(part 1 of 2)
# Autodesk Inventor assembly: Motedius_QR-500
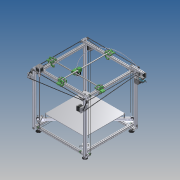
[picture p0: Inventor's stored thumbnail of the model, 180x180]
Saved by Autodesk Inventor 2015 SP1 (Build 190203100, 203)
## iProperties
Created: 2015-01-08
Part Number: Motedius_QR-500
Document SubType Name: Assembly
Designer: Marc
Author: Marc
## Documents named in this file (64)
- E:\Modellflieger\3D Drucker\MotediusQR 500mm\Motedius_QR-500.iam
- E:\Modellflieger\3D Drucker\MotediusQR 500mm\Motedius_20x20_B-Type_Slot-6_500.ipt
- E:\Modellflieger\3D Drucker\MotediusQR 500mm\Motedius_20x20_B-Type_Slot-6_500_MIR.ipt
- E:\Modellflieger\3D Drucker\Eigene Teile\Nema17 Schrittmotor\Nema17_Schrittmotor.iam
- E:\Modellflieger\3D Drucker\Eigene Teile\Nema17 Schrittmotor\Nema17_Montageplatte.ipt
- C:\Users\Marc\Documents\Inventor\Content Center Files\R2015\de-DE\DIN 84\DIN 84 - M3 x 6.ipt
- C:\Users\Marc\Documents\Inventor\Content Center Files\R2015\de-DE\DIN 934\DIN 934 - M6 x 1.ipt
- C:\Users\Marc\Documents\Inventor\Content Center Files\R2015\de-DE\DIN 125-1  A\DIN 125 - A 6,4.ipt
- C:\Users\Marc\Documents\Inventor\Content Center Files\R2015\de-DE\DIN 84\DIN 84 - M6 x 50.ipt
- E:\Modellflieger\3D Drucker\Eigene Teile\Motedis 20 B-Typ Nut 6 Parts\Motedius Gelenkfuß 10 PA\Motedius_Gelenkfuß_10_PA_M6x60.iam
- E:\Modellflieger\3D Drucker\MotediusQR 500mm\Motedius_20x20_B-Type_Slot-6_600.ipt
- E:\Modellflieger\3D Drucker\MotediusQR 500mm\Motedius_20x20_B-Type_Slot-6_290.ipt
- E:\Modellflieger\3D Drucker\MotediusQR 500mm\10mm_Alu_Linearwelle_500mm.ipt
- E:\Modellflieger\3D Drucker\MotediusQR 500mm\X_Y_mit_LM10UU\Lagerblock_Lm10UU.ipt
- E:\Modellflieger\3D Drucker\Eigene Teile\LinearWagen_Mauro_Wheels\Mauro_Wagen_QR_version.iam
- E:\Modellflieger\3D Drucker\Eigene Teile\Linearlager_LM10UU.ipt
- E:\Modellflieger\3D Drucker\Eigene Teile\Openbuilds_Dual_V-Wheel\Openbuilds_Dual_V-Wheel.iam
- E:\Modellflieger\3D Drucker\Eigene Teile\Motedis 20 B-Typ Nut 6 Parts\Motedis_Winkel.ipt
- C:\Users\Marc\Documents\Inventor\Content Center Files\R2015\de-DE\DIN 934\DIN 934 - M5 x 0,8.ipt
- E:\Modellflieger\3D Drucker\Eigene Teile\GT2_20tooth_Pulley\GT2_20tooth.ipt
- E:\Modellflieger\3D Drucker\Eigene Teile\Eigene Schrauben\QR_Ramenschraube_unten_M6x60.iam
- E:\Modellflieger\3D Drucker\Eigene Teile\Eigene Schrauben\QR_Rahmenschraube_oben_M6x80.iam
- E:\Modellflieger\3D Drucker\Eigene Teile\Seilrolle druckbar\Seilrolle.iam
- C:\Users\Marc\Documents\Inventor\Content Center Files\R2015\de-DE\DIN 9021\DIN 9021 - 6,4.ipt
- E:\Modellflieger\3D Drucker\Eigene Teile\Seilrolle druckbar\Distanzscheibe_6x10x0,5mm.ipt
- E:\Modellflieger\3D Drucker\MotediusQR 500mm\Motedius_QR-500\Konstruktions-Assistent\Übertragung des Zahnriemens1.iam
- E:\Modellflieger\3D Drucker\MotediusQR 500mm\Motedius_QR-500\Konstruktions-Assistent\Übertragung des Zahnriemens2.iam
- E:\Modellflieger\3D Drucker\MotediusQR 500mm\Motedius_QR-500\Konstruktions-Assistent\Übertragung des Zahnriemens3.iam
- E:\Modellflieger\3D Drucker\MotediusQR 500mm\Motedius_QR-500\Konstruktions-Assistent\Übertragung des Zahnriemens4.iam
- E:\Modellflieger\3D Drucker\Eigene Teile\Nema17 Schrittmotor\Nema17_Montageplatte_Z-Achse.ipt
- C:\Users\Marc\Documents\Inventor\Content Center Files\R2015\de-DE\DIN 9021\DIN 9021 - 5,3.ipt
- E:\Modellflieger\3D Drucker\MotediusQR 500mm\Importierte Komponenten\Wellenkupplung5-8mm\Wellenkupplung5-8mm.iam
- E:\Modellflieger\3D Drucker\Eigene Teile\Gewindestange_M8x420mm.ipt
- E:\Modellflieger\3D Drucker\MotediusQR 500mm\Gewindestück_M5_Z-Achse.ipt
- E:\Modellflieger\3D Drucker\MotediusQR 500mm\Z-Stage_Wheel_plate.ipt
- E:\Modellflieger\3D Drucker\MotediusQR 500mm\Z-Stage_Wheel_plate_20x20.ipt
- C:\Users\Marc\Documents\Inventor\Content Center Files\R2015\de-DE\DIN 84\DIN 84 - M5 x 30.ipt
- E:\Modellflieger\3D Drucker\Eigene Teile\Eigene Schrauben\Ösenschraube_M3x15.ipt
- C:\Users\Marc\Documents\Inventor\Content Center Files\R2015\de-DE\DIN 934\DIN 934 - M3 x 0,5.ipt
- C:\Users\Marc\Documents\Inventor\Content Center Files\R2015\de-DE\DIN 84\DIN 84 - M5 x 6.ipt
- C:\Users\Marc\Documents\Inventor\Content Center Files\R2015\de-DE\DIN 84\DIN 84 - M5 x 8.ipt
- C:\Users\Marc\Documents\Inventor\Content Center Files\R2015\de-DE\DIN 934\DIN 934 - M8 x 1,25.ipt
- E:\Modellflieger\3D Drucker\MotediusQR 500mm\Z_Stage_Nut_holder_15x15alu.ipt
- C:\Users\Marc\Documents\Inventor\Content Center Files\R2015\de-DE\DIN 84\DIN 84 - M5 x 20.ipt
- E:\Modellflieger\3D Drucker\MotediusQR 500mm\Aluplatte_5mm.ipt
- C:\Users\Marc\Documents\Inventor\Content Center Files\R2015\de-DE\DIN 84\DIN 84 - M5 x 40.ipt
- E:\Modellflieger\3D Drucker\MotediusQR 500mm\Seil1.ipt
- E:\Modellflieger\3D Drucker\MotediusQR 500mm\Seil2.ipt
- E:\Modellflieger\3D Drucker\MotediusQR 500mm\Seil-3.ipt
- E:\Modellflieger\3D Drucker\MotediusQR 500mm\Gewindestück_M5_Z-Achse_55mm.ipt
- E:\Modellflieger\3D Drucker\Eigene Teile\Motedis 20 B-Typ Nut 6 Parts\Motedius_20x20_B-Type_Slot-6_120.ipt
- Motedius_20x20_B-Type_Slot-6_120.ipt
- E:\Modellflieger\3D Drucker\Eigene Teile\POM Extruder\extruder_180Grad.iam
- E:\Modellflieger\3D Drucker\Eigene Teile\Eigene Schrauben\DIN 84 - M6 x 70.ipt
- C:\Users\Marc\Documents\Inventor\Content Center Files\R2015\de-DE\DIN 84\DIN 84 - M5 x 10.ipt
- E:\Modellflieger\3D Drucker\MotediusQR 500mm\Importierte Komponenten\E3D_V6_1.75mm_Universal_HotEnd_Mockup\E3D_V6_1.75mm_Universal_HotEnd_Mockup.ipt
- E:\Modellflieger\3D Drucker\MotediusQR 500mm\Importierte Komponenten\E3D_V6_Fan_Duct\E3D_V6_Fan_Duct.ipt
- E:\Modellflieger\3D Drucker\MotediusQR 500mm\PTFE_Tube_4x2.ipt
- E:\Modellflieger\3D Drucker\MotediusQR 500mm\Importierte Komponenten\12VDC-1.1875-X-0.375-DELTA-BOX-FAN\12VDC-1.1875-X-0.375-DELTA-BOX-FAN.ipt
- C:\Users\Marc\Documents\Inventor\Content Center Files\R2015\de-DE\DIN 84\DIN 84 - M3 x 10.ipt
- C:\Users\Marc\Documents\Inventor\Content Center Files\R2015\de-DE\DIN 84\DIN 84 - M3 x 22.ipt
- C:\Users\Marc\Documents\Inventor\Content Center Files\R2015\de-DE\DIN 84\DIN 84 - M3 x 18.ipt
- E:\Modellflieger\3D Drucker\Eigene Teile\gt2-belt-clamps\gt2_clip_v2.ipt
- C:\Users\Marc\Documents\Inventor\Content Center Files\R2015\de-DE\DIN 84\DIN 84 - M3 x 14.ipt
## Components (294 placed, 59 different names)
1. Motedius_20x20_B-Type_Slot-6_500:1 — Tangential:1, Fluchtend:1, Passend:1, Tangential:3, Fluchtend:3, Passend:3, Passend:5, Passend:7, Passend:9, Passend:79, Passend:89, Fluchtend:55
2. Motedius_20x20_B-Type_Slot-6_500:2 — Tangential:1, Fluchtend:1, Passend:1, Tangential:2, Passend:2, Fluchtend:2, Fluchtend:5, Passend:10, Passend:13, Fluchtend:7, Einfügen:30, Einfügen:32, Fluchtend:44
3. Motedius_20x20_B-Type_Slot-6_500:3 — Tangential:2, Passend:2, Fluchtend:2, Passend:11, Passend:14, Passend:91, Passend:93, Passend:137, Fluchtend:45
4. Motedius_20x20_B-Type_Slot-6_500:4 — Tangential:3, Fluchtend:3, Passend:3, Passend:4, Passend:6, Fluchtend:4, Passend:8, Passend:12, Fluchtend:6, Einfügen:29, Einfügen:31, Fluchtend:31, Fluchtend:54
5. Motedius_20x20_B-Type_Slot-6_500:5 — Passend:7, Fluchtend:4, Passend:8, Passend:20, Fluchtend:12, Einfügen:71, Einfügen:72, Einfügen:86, Einfügen:87
6. Motedius_20x20_B-Type_Slot-6_500:6 — Passend:9, Fluchtend:5, Passend:10, Passend:23, Fluchtend:13, Einfügen:76, Einfügen:77, Einfügen:79, Einfügen:80
7. Motedius_20x20_B-Type_Slot-6_500:7 — Passend:13, Passend:14, Fluchtend:7, Passend:25, Fluchtend:14, Einfügen:75, Einfügen:78
8. Motedius_20x20_B-Type_Slot-6_500:8 — Passend:11, Passend:12, Fluchtend:6, Passend:27, Fluchtend:15, Einfügen:73, Einfügen:74, Einfügen:88, Einfügen:89
9. Motedius_20x20_B-Type_Slot-6_500_MIR:1 — Passend:15, Passend:16, Fluchtend:8, Tangential:4, Passend:19, Fluchtend:11, Tangential:6, Passend:21, Passend:22, Einfügen:26, Einfügen:27, Passend:163, Passend:164
10. Motedius_20x20_B-Type_Slot-6_500_MIR:2 — Passend:16, Fluchtend:8, Tangential:4, Fluchtend:9, Passend:17, Tangential:5, Passend:67, Passend:165, Passend:166, Passend:262, Fluchtend:62, Passend:263
11. Motedius_20x20_B-Type_Slot-6_500_MIR:3 — Fluchtend:9, Passend:17, Tangential:5, Passend:24, Passend:26, Einfügen:25, Einfügen:28, Passend:159, Passend:160
12. Motedius_20x20_B-Type_Slot-6_500_MIR:4 — Passend:18, Fluchtend:10, Passend:19, Fluchtend:11, Tangential:6, Passend:63, Passend:65, Passend:161, Passend:162, Passend:175, Fluchtend:34, Fluchtend:35
13. Nema17_Schrittmotor:1 [sub-assembly] — Einfügen:1, Tangential:7, Einfügen:2, Einfügen:3, Einfügen:4, Einfügen:5, Einfügen:66
14. Nema17_Montageplatte:1 — Einfügen:1, Tangential:7, Passend:20, Fluchtend:12, Passend:21
15. DIN 84 - ersetzt durch DIN EN ISO 1207 M3 x 6:1 — Einfügen:2
16. DIN 84 - ersetzt durch DIN EN ISO 1207 M3 x 6:2 — Einfügen:5
17. DIN 84 - ersetzt durch DIN EN ISO 1207 M3 x 6:3 — Einfügen:3
18. DIN 84 - ersetzt durch DIN EN ISO 1207 M3 x 6:4 — Einfügen:4
19. Nema17_Schrittmotor:2 [sub-assembly] — Einfügen:67
20. Nema17_Montageplatte:2 — Passend:22, Passend:23, Fluchtend:13
21. DIN 84 - ersetzt durch DIN EN ISO 1207 M3 x 6:5
22. DIN 84 - ersetzt durch DIN EN ISO 1207 M3 x 6:6
23. DIN 84 - ersetzt durch DIN EN ISO 1207 M3 x 6:7
24. DIN 84 - ersetzt durch DIN EN ISO 1207 M3 x 6:8
25. Nema17_Schrittmotor:3 [sub-assembly] — Einfügen:68
26. Nema17_Montageplatte:3 — Passend:24, Passend:25, Fluchtend:14
27. DIN 84 - ersetzt durch DIN EN ISO 1207 M3 x 6:9
28. DIN 84 - ersetzt durch DIN EN ISO 1207 M3 x 6:10
29. DIN 84 - ersetzt durch DIN EN ISO 1207 M3 x 6:11
30. DIN 84 - ersetzt durch DIN EN ISO 1207 M3 x 6:12
31. Nema17_Schrittmotor:4 [sub-assembly] — Einfügen:65
32. Nema17_Montageplatte:4 — Passend:26, Passend:27, Fluchtend:15
33. DIN 84 - ersetzt durch DIN EN ISO 1207 M3 x 6:13
34. DIN 84 - ersetzt durch DIN EN ISO 1207 M3 x 6:14
35. DIN 84 - ersetzt durch DIN EN ISO 1207 M3 x 6:15
36. DIN 84 - ersetzt durch DIN EN ISO 1207 M3 x 6:16
37. DIN 84 - ersetzt durch DIN EN ISO 1207 M6 x 50:1 — Passend:52, Passend:53, Passend:62, Passend:70
38. DIN 125-1 A A 6,4:9 — Passend:52, Passend:53, Einfügen:25
39. DIN 84 - M6 x 70:1 — Passend:265, Passend:267
40. DIN 125-1 A A 6,4:10 — Einfügen:28
41. DIN 84 - ersetzt durch DIN EN ISO 1207 M6 x 50:3 — Passend:64, Passend:72
42. DIN 125-1 A A 6,4:11 — Einfügen:26
43. DIN 84 - ersetzt durch DIN EN ISO 1207 M6 x 50:4 — Passend:66, Passend:74
44. DIN 125-1 A A 6,4:12 — Einfügen:27
45. DIN 125-1 A A 6,4:14 — Passend:62, Passend:63, Passend:71
46. DIN 125-1 A A 6,4:15 — Passend:64, Passend:65, Passend:73
47. DIN 125-1 A A 6,4:16 — Passend:66, Passend:67, Passend:75
48. DIN 934 - ersetzt durch DIN EN 24032/28673/28674 M6:6 — Passend:70, Passend:71
49. DIN 934 - ersetzt durch DIN EN 24032/28673/28674 M6:7 — Passend:72, Passend:73
50. DIN 934 - ersetzt durch DIN EN 24032/28673/28674 M6:8 — Passend:74, Passend:75
51. Motedius_Gelenkfuß_10_PA_M6x60:1 [sub-assembly] — Passend:76, Passend:77, Passend:78, Passend:80
52. DIN 125-1 A A 6,4:17 — Passend:76, Passend:77, Einfügen:29
53. DIN 125-1 A A 6,4:18 — Passend:78, Passend:79, Passend:81
54. DIN 934 - ersetzt durch DIN EN 24032/28673/28674 M6:9 — Passend:80, Passend:81
55. Motedius_Gelenkfuß_10_PA_M6x60:2 [sub-assembly] — Passend:88, Passend:94
56. DIN 125-1 A A 6,4:19 — Einfügen:30
57. Motedius_Gelenkfuß_10_PA_M6x60:3 [sub-assembly] — Passend:92, Passend:98
58. DIN 125-1 A A 6,4:20 — Einfügen:31
59. Motedius_Gelenkfuß_10_PA_M6x60:4 [sub-assembly] — Passend:90, Passend:96
60. DIN 125-1 A A 6,4:21 — Einfügen:32
61. DIN 125-1 A A 6,4:22 — Passend:88, Passend:89, Passend:95
62. DIN 125-1 A A 6,4:23 — Passend:90, Passend:91, Passend:97
63. DIN 125-1 A A 6,4:24 — Passend:92, Passend:93, Passend:99
64. DIN 934 - ersetzt durch DIN EN 24032/28673/28674 M6:10 — Passend:94, Passend:95
65. DIN 934 - ersetzt durch DIN EN 24032/28673/28674 M6:11 — Passend:96, Passend:97
66. DIN 934 - ersetzt durch DIN EN 24032/28673/28674 M6:12 — Passend:98, Passend:99
67. Motedius_20x20_B-Type_Slot-6_600:1 — Passend:135, Fluchtend:23, Fluchtend:24, Fluchtend:25, Passend:136, Fluchtend:26, Passend:137, Fluchtend:27, Passend:138, Passend:141, Passend:142, Passend:144, Fluchtend:29, Passend:196, Fluchtend:40, Fluchtend:41, Fluchtend:42, Passend:197, Passend:202, Fluchtend:46, Fluchtend:47, Passend:203, Fluchtend:48, Passend:235, Passend:237, Passend:243
68. Motedius_20x20_B-Type_Slot-6_290:1 — Passend:135, Fluchtend:23, Fluchtend:24, Passend:140, Passend:145, Passend:186, Fluchtend:36, Fluchtend:37, Passend:187, Fluchtend:38, Fluchtend:39, Passend:232, Passend:241
69. Motedius_20x20_B-Type_Slot-6_290:2 — Fluchtend:25, Passend:136, Fluchtend:26, Passend:139, Passend:143, Fluchtend:28, Fluchtend:50, Passend:210, Fluchtend:51, Passend:211, Fluchtend:52, Passend:239
70. Openbuilds_Dual_V-Wheel:5 [sub-assembly] — Einfügen:155
71. Openbuilds_Dual_V-Wheel:6 [sub-assembly] — Einfügen:153
72. Openbuilds_Dual_V-Wheel:7 [sub-assembly] — Einfügen:157
73. Openbuilds_Dual_V-Wheel:8 [sub-assembly] — Einfügen:150
74. Motedis_Winkel:9 — Fluchtend:27, Passend:138, Passend:139, Fluchtend:45, Einfügen:179, Einfügen:180
75. Motedis_Winkel:10 — Passend:140, Passend:141, Fluchtend:31, Einfügen:177, Einfügen:178
76. Motedis_Winkel:11 — Passend:142, Passend:143, Fluchtend:28, Fluchtend:44, Einfügen:181, Einfügen:182
77. Motedis_Winkel:12 — Passend:144, Passend:145, Fluchtend:29, Einfügen:183, Einfügen:184
78. Mauro_Wagen_QR_version:5 [sub-assembly] — Passend:159, Passend:160, Fluchtend:33, Passend:289, Fluchtend:73, Fluchtend:74, Einfügen:203
79. Mauro_Wagen_QR_version:6 [sub-assembly] — Passend:161, Passend:162, Fluchtend:32, Passend:287, Fluchtend:69, Fluchtend:70, Einfügen:204
80. Mauro_Wagen_QR_version:7 [sub-assembly] — Passend:165, Passend:166, Fluchtend:32, Einfügen:48, Passend:288, Fluchtend:71, Fluchtend:72, Einfügen:206
81. Mauro_Wagen_QR_version:8 [sub-assembly] — Passend:163, Passend:164, Fluchtend:33, Einfügen:47, Passend:285, Fluchtend:67, Fluchtend:68, Passend:286, Einfügen:205
82. 10mm_Alu_Linearwelle_500mm:1 — Einfügen:47, Einfügen:52
83. 10mm_Alu_Linearwelle_500mm:2 — Einfügen:48, Einfügen:51
84. Lagerblock_Lm10UU:1 — Einfügen:49, Einfügen:50, Einfügen:51, Einfügen:52, Einfügen:195, Einfügen:197, Einfügen:198, Passend:274, Passend:276, Einfügen:199, Einfügen:200, Passend:278, Passend:280, Einfügen:201, Einfügen:202, Passend:282, Passend:284
85. Linearlager_LM10UU:1 — Einfügen:50
86. Linearlager_LM10UU:2 — Einfügen:49
87. QR_Rahmenschraube_oben_M6x80:2 [sub-assembly] — Einfügen:75
88. QR_Rahmenschraube_oben_M6x80:3 [sub-assembly] — Einfügen:72
89. QR_Rahmenschraube_oben_M6x80:4 [sub-assembly] — Einfügen:73
90. QR_Rahmenschraube_oben_M6x80:5 [sub-assembly] — Einfügen:77, Einfügen:111
91. QR_Rahmenschraube_oben_M6x80:6 [sub-assembly] — Einfügen:74, Einfügen:135
92. QR_Rahmenschraube_oben_M6x80:7 [sub-assembly] — Einfügen:76
93. QR_Rahmenschraube_oben_M6x80:8 [sub-assembly] — Einfügen:71
94. DIN 84 - ersetzt durch DIN EN ISO 1207 M5 x 30:2 — Einfügen:156, Passend:212, Passend:214, Passend:216
95. DIN 84 - ersetzt durch DIN EN ISO 1207 M5 x 30:1 — Passend:169, Einfügen:151, Passend:198, Passend:200
96. DIN 934 - ersetzt durch DIN EN 24032/28673/28674 M5:2 — Passend:169, Einfügen:152
97. GT2_20tooth:1 — Einfügen:65
98. GT2_20tooth:2 — Einfügen:66
99. GT2_20tooth:3 — Einfügen:67
100. GT2_20tooth:4 — Einfügen:68
101. QR_Ramenschraube_unten_M6x60:1 [sub-assembly] — Einfügen:147
102. QR_Rahmenschraube_oben_M6x80:1 [sub-assembly] — Einfügen:148
103. QR_Ramenschraube_unten_M6x60:2 [sub-assembly] — Einfügen:78
104. QR_Ramenschraube_unten_M6x60:3 [sub-assembly] — Einfügen:80
105. QR_Ramenschraube_unten_M6x60:4 [sub-assembly] — Einfügen:79, Einfügen:81, Passend:176
106. Seilrolle:1 [sub-assembly] — Einfügen:83, Einfügen:84
107. DIN 9021 6,4:1 — Einfügen:81, Einfügen:82
108. DIN 9021 6,4:2 — Einfügen:85, Passend:177
109. Distanzscheibe_6x10x0,5mm:1 — Einfügen:82, Einfügen:83
110. Distanzscheibe_6x10x0,5mm:2 — Einfügen:84, Einfügen:85
111. QR_Ramenschraube_unten_M6x60:5 [sub-assembly] — Einfügen:87, Einfügen:123
112. QR_Ramenschraube_unten_M6x60:6 [sub-assembly] — Einfügen:86, Einfügen:117
113. QR_Ramenschraube_unten_M6x60:7 [sub-assembly] — Einfügen:89, Einfügen:129
114. QR_Ramenschraube_unten_M6x60:8 [sub-assembly] — Einfügen:88, Einfügen:141
115. Übertragung des Zahnriemens:1 [sub-assembly]
116. Übertragung des Zahnriemens:2 [sub-assembly]
117. Übertragung des Zahnriemens:3 [sub-assembly]
118. Übertragung des Zahnriemens:4 [sub-assembly]
119. Nema17_Schrittmotor:5 [sub-assembly] — Einfügen:99
120. Nema17_Montageplatte_Z-Achse:1 — Passend:175, Fluchtend:34, Fluchtend:35, Einfügen:95, Einfügen:97, Einfügen:193, Einfügen:194
121. DIN 84 - ersetzt durch DIN EN ISO 1207 M3 x 6:17
122. DIN 84 - ersetzt durch DIN EN ISO 1207 M3 x 6:18
123. DIN 84 - ersetzt durch DIN EN ISO 1207 M3 x 6:19
124. DIN 84 - ersetzt durch DIN EN ISO 1207 M3 x 6:20
125. DIN 9021 5,3:1 — Einfügen:95, Einfügen:96
126. DIN 9021 5,3:2 — Einfügen:96
127. DIN 9021 5,3:3 — Einfügen:98
128. DIN 9021 5,3:4 — Einfügen:97, Einfügen:98
129. Wellenkupplung5-8mm:1 [sub-assembly] — Einfügen:99, Einfügen:100
130. Gewindestange_M8x420mm:1 — Einfügen:100, Tangential:12
131. DIN 934 - ersetzt durch DIN EN 24032/28673/28674 M6:13 — Passend:176, Passend:177
132. Seilrolle:2 [sub-assembly]
133. DIN 9021 6,4:3 — Einfügen:111
134. DIN 9021 6,4:4 — Einfügen:105
135. Distanzscheibe_6x10x0,5mm:3
136. Distanzscheibe_6x10x0,5mm:4
137. DIN 934 - ersetzt durch DIN EN 24032/28673/28674 M6:14 — Einfügen:105
138. Seilrolle:3 [sub-assembly]
139. DIN 9021 6,4:5 — Einfügen:117
140. DIN 9021 6,4:6
141. Distanzscheibe_6x10x0,5mm:5
142. Distanzscheibe_6x10x0,5mm:6
143. DIN 934 - ersetzt durch DIN EN 24032/28673/28674 M6:15
144. Seilrolle:4 [sub-assembly] — Fluchtend:56
145. DIN 9021 6,4:7 — Einfügen:123
146. DIN 9021 6,4:8
147. Distanzscheibe_6x10x0,5mm:7
148. Distanzscheibe_6x10x0,5mm:8
149. DIN 934 - ersetzt durch DIN EN 24032/28673/28674 M6:16
150. Seilrolle:5 [sub-assembly]
151. DIN 9021 6,4:9 — Einfügen:129
152. DIN 9021 6,4:10
153. Distanzscheibe_6x10x0,5mm:9
154. Distanzscheibe_6x10x0,5mm:10
155. DIN 934 - ersetzt durch DIN EN 24032/28673/28674 M6:17
156. Seilrolle:6 [sub-assembly]
157. DIN 9021 6,4:11 — Einfügen:135
158. DIN 9021 6,4:12
159. Distanzscheibe_6x10x0,5mm:11
160. Distanzscheibe_6x10x0,5mm:12
161. DIN 934 - ersetzt durch DIN EN 24032/28673/28674 M6:18
162. Seilrolle:7 [sub-assembly] — Fluchtend:59
163. DIN 9021 6,4:13 — Einfügen:141
164. DIN 9021 6,4:14
165. Distanzscheibe_6x10x0,5mm:13
166. Distanzscheibe_6x10x0,5mm:14
167. DIN 934 - ersetzt durch DIN EN 24032/28673/28674 M6:19
168. Seilrolle:8 [sub-assembly]
169. DIN 9021 6,4:15 — Einfügen:147
170. DIN 9021 6,4:16
171. Distanzscheibe_6x10x0,5mm:15
172. Distanzscheibe_6x10x0,5mm:16
173. DIN 934 - ersetzt durch DIN EN 24032/28673/28674 M6:20
174. Seilrolle:9 [sub-assembly]
175. DIN 9021 6,4:17 — Einfügen:148
176. DIN 9021 6,4:18
177. Distanzscheibe_6x10x0,5mm:17
178. Distanzscheibe_6x10x0,5mm:18
179. DIN 934 - ersetzt durch DIN EN 24032/28673/28674 M6:21
180. Gewindestück_M5_Z-Achse:1 — Einfügen:149, Passend:188, Passend:190, Passend:192, Passend:194
181. Z-Stage_Wheel_plate:1 — Passend:186, Fluchtend:36, Fluchtend:37, Einfügen:149, Einfügen:150, Passend:189, Passend:193, Einfügen:173, Einfügen:174
182. Z-Stage_Wheel_plate:2 — Passend:187, Fluchtend:38, Fluchtend:39, Passend:191, Passend:195, Einfügen:171, Einfügen:172
183. DIN 934 - ersetzt durch DIN EN 24032/28673/28674 M5:5 — Passend:188, Passend:189
184. DIN 934 - ersetzt durch DIN EN 24032/28673/28674 M5:6 — Passend:190, Passend:191
185. DIN 934 - ersetzt durch DIN EN 24032/28673/28674 M5:7 — Passend:192, Passend:193
186. DIN 934 - ersetzt durch DIN EN 24032/28673/28674 M5:8 — Passend:194, Passend:195
187. Z-Stage_Wheel_plate_20x20:1 — Fluchtend:42, Passend:197, Fluchtend:43, Einfügen:152, Passend:201, Einfügen:169, Einfügen:170
188. Z-Stage_Wheel_plate_20x20:2 — Passend:196, Fluchtend:40, Fluchtend:41, Fluchtend:43, Einfügen:151, Einfügen:153, Passend:199, Einfügen:158, Passend:219, Passend:221, Einfügen:167, Einfügen:168
189. DIN 934 - ersetzt durch DIN EN 24032/28673/28674 M5:9 — Passend:198, Passend:199
190. DIN 934 - ersetzt durch DIN EN 24032/28673/28674 M5:10 — Passend:200, Passend:201
191. Z-Stage_Wheel_plate_20x20:3 — Passend:202, Fluchtend:46, Fluchtend:47, Fluchtend:49, Passend:205, Einfügen:159, Passend:227, Passend:229, Einfügen:161, Einfügen:162, Einfügen:192, Passend:261
192. Z-Stage_Wheel_plate:3 — Passend:203, Fluchtend:48, Fluchtend:49, Einfügen:155, Passend:207, Passend:209, Einfügen:175, Einfügen:176
193. Gewindestück_M5_Z-Achse_55mm:1 — Einfügen:192, Passend:260
194. DIN 934 - ersetzt durch DIN EN 24032/28673/28674 M5:11 — Passend:205
195. DIN 934 - ersetzt durch DIN EN 24032/28673/28674 M5:12 — Passend:207
196. DIN 934 - ersetzt durch DIN EN 24032/28673/28674 M5:13 — Passend:209
197. Z-Stage_Wheel_plate_20x20:4 — Fluchtend:50, Passend:210, Fluchtend:51, Fluchtend:53, Einfügen:156, Einfügen:157, Passend:215, Einfügen:160, Passend:223, Passend:225, Einfügen:165, Einfügen:166
198. Z-Stage_Wheel_plate_20x20:5 — Passend:211, Fluchtend:52, Fluchtend:53, Passend:213, Passend:217, Einfügen:163, Einfügen:164
199. DIN 934 - ersetzt durch DIN EN 24032/28673/28674 M5:14 — Passend:212, Passend:213
200. DIN 934 - ersetzt durch DIN EN 24032/28673/28674 M5:15 — Passend:214, Passend:215
201. DIN 934 - ersetzt durch DIN EN 24032/28673/28674 M5:16 — Passend:216, Passend:217
202. Ösenschraube_M3x15:1 — Einfügen:158, Passend:218, Passend:220
203. DIN 934 - ersetzt durch DIN EN 24032/28673/28674 M3:1 — Passend:218, Passend:219
204. DIN 934 - ersetzt durch DIN EN 24032/28673/28674 M3:2 — Passend:220, Passend:221
205. Ösenschraube_M3x15:2 — Einfügen:159, Passend:226, Passend:228
206. Ösenschraube_M3x15:3 — Einfügen:160, Passend:222, Passend:224
207. DIN 934 - ersetzt durch DIN EN 24032/28673/28674 M3:3 — Passend:222, Passend:223
208. DIN 934 - ersetzt durch DIN EN 24032/28673/28674 M3:4 — Passend:224, Passend:225
209. DIN 934 - ersetzt durch DIN EN 24032/28673/28674 M3:5 — Passend:226, Passend:227
210. DIN 934 - ersetzt durch DIN EN 24032/28673/28674 M3:6 — Passend:228, Passend:229
211. DIN 84 - ersetzt durch DIN EN ISO 1207 M5 x 6:1 — Einfügen:161
212. DIN 84 - ersetzt durch DIN EN ISO 1207 M5 x 6:2 — Einfügen:162
213. DIN 84 - ersetzt durch DIN EN ISO 1207 M5 x 6:3 — Einfügen:164
214. DIN 84 - ersetzt durch DIN EN ISO 1207 M5 x 6:4 — Einfügen:163
215. DIN 84 - ersetzt durch DIN EN ISO 1207 M5 x 6:5 — Einfügen:165
216. DIN 84 - ersetzt durch DIN EN ISO 1207 M5 x 6:6 — Einfügen:166
217. DIN 84 - ersetzt durch DIN EN ISO 1207 M5 x 6:7 — Einfügen:167
218. DIN 84 - ersetzt durch DIN EN ISO 1207 M5 x 6:8 — Einfügen:168
219. DIN 84 - ersetzt durch DIN EN ISO 1207 M5 x 6:9 — Einfügen:169
220. DIN 84 - ersetzt durch DIN EN ISO 1207 M5 x 6:10 — Einfügen:170
221. DIN 84 - ersetzt durch DIN EN ISO 1207 M5 x 6:11 — Einfügen:171
222. DIN 84 - ersetzt durch DIN EN ISO 1207 M5 x 6:12 — Einfügen:172
223. DIN 84 - ersetzt durch DIN EN ISO 1207 M5 x 6:13 — Einfügen:173
224. DIN 84 - ersetzt durch DIN EN ISO 1207 M5 x 6:14 — Einfügen:174
225. DIN 84 - ersetzt durch DIN EN ISO 1207 M5 x 6:15 — Einfügen:175
226. DIN 84 - ersetzt durch DIN EN ISO 1207 M5 x 6:16 — Einfügen:176
227. DIN 84 - ersetzt durch DIN EN ISO 1207 M5 x 8:1 — Einfügen:178
228. DIN 84 - ersetzt durch DIN EN ISO 1207 M5 x 8:2 — Einfügen:177
229. DIN 84 - ersetzt durch DIN EN ISO 1207 M5 x 8:3 — Einfügen:179
230. DIN 84 - ersetzt durch DIN EN ISO 1207 M5 x 8:4 — Einfügen:180
231. DIN 84 - ersetzt durch DIN EN ISO 1207 M5 x 8:5 — Einfügen:181
232. DIN 84 - ersetzt durch DIN EN ISO 1207 M5 x 8:6 — Einfügen:182
233. DIN 84 - ersetzt durch DIN EN ISO 1207 M5 x 8:7 — Einfügen:183
234. DIN 84 - ersetzt durch DIN EN ISO 1207 M5 x 8:8 — Einfügen:184
235. DIN 934 - ersetzt durch DIN EN 24032/28673/28674 M8:1 — Einfügen:185, Passend:230, Tangential:12
236. Z_Stage_Nut_holder_15x15alu:1 — Einfügen:185, Passend:230, Einfügen:186, Passend:231, Passend:232, Einfügen:187
237. DIN 934 - ersetzt durch DIN EN 24032/28673/28674 M8:2 — Einfügen:186, Passend:231
238. DIN 84 - ersetzt durch DIN EN ISO 1207 M5 x 20:1 — Passend:233, Passend:234
239. DIN 9021 5,3:5 — Passend:233, Passend:234, Einfügen:187
240. Aluplatte_5mm:1 — Einfügen:188, Einfügen:189, Einfügen:190, Einfügen:191, Fluchtend:54, Fluchtend:55, Passend:253, Passend:255, Passend:257, Passend:259
241. DIN 84 - ersetzt durch DIN EN ISO 1207 M5 x 40:2 — Einfügen:189, Passend:238, Passend:250, Passend:256
242. DIN 84 - ersetzt durch DIN EN ISO 1207 M5 x 40:3 — Einfügen:188, Passend:235, Passend:236, Passend:244, Passend:258
243. DIN 84 - ersetzt durch DIN EN ISO 1207 M5 x 40:4 — Einfügen:190, Passend:240, Passend:248, Passend:252
244. DIN 84 - ersetzt durch DIN EN ISO 1207 M5 x 40:5 — Einfügen:191, Passend:242, Passend:246, Passend:254
245. DIN 9021 5,3:6 — Passend:236, Passend:237, Passend:245
246. DIN 9021 5,3:7 — Passend:238, Passend:239, Passend:251
247. DIN 9021 5,3:8 — Passend:240, Passend:241, Passend:249
248. DIN 9021 5,3:9 — Passend:242, Passend:243, Passend:247
249. DIN 934 - ersetzt durch DIN EN 24032/28673/28674 M5:17 — Passend:244, Passend:245
250. DIN 934 - ersetzt durch DIN EN 24032/28673/28674 M5:18 — Passend:246, Passend:247
251. DIN 934 - ersetzt durch DIN EN 24032/28673/28674 M5:19 — Passend:248, Passend:249
252. DIN 934 - ersetzt durch DIN EN 24032/28673/28674 M5:20 — Passend:250, Passend:251
253. DIN 934 - ersetzt durch DIN EN 24032/28673/28674 M5:21 — Passend:252, Passend:253
254. DIN 934 - ersetzt durch DIN EN 24032/28673/28674 M5:22 — Passend:254, Passend:255
255. DIN 934 - ersetzt durch DIN EN 24032/28673/28674 M5:23 — Passend:256, Passend:257
256. DIN 934 - ersetzt durch DIN EN 24032/28673/28674 M5:24 — Passend:258, Passend:259
257. Seil1:1
258. Seil2:1 — Fluchtend:57, Fluchtend:58
259. Seil-3:1 — Fluchtend:60, Fluchtend:61
260. DIN 934 - ersetzt durch DIN EN 24032/28673/28674 M5:25 — Passend:260, Passend:261
261. Motedius_20x20_B-Type_Slot-6_120:1 — Passend:262, Fluchtend:62, Passend:263, Passend:264, Fluchtend:63, Fluchtend:64, Passend:266
262. extruder_180Grad:1 [sub-assembly] — Passend:264, Fluchtend:63, Fluchtend:64, Passend:270
263. DIN 9021 6,4:19 — Passend:265, Passend:266, Passend:268
264. DIN 934 - ersetzt durch DIN EN 24032/28673/28674 M6:22 — Passend:267, Passend:268
265. DIN 84 - ersetzt durch DIN EN ISO 1207 M5 x 10:1 — Einfügen:193
266. DIN 84 - ersetzt durch DIN EN ISO 1207 M5 x 10:2 — Einfügen:194
267. E3D_V6_1.75mm_Universal_HotEnd_Mockup:1 — Einfügen:195, Tangential:13, Passend:269, Fluchtend:66
268. E3D_V6_Fan_Duct:1 — Tangential:13, Einfügen:196
269. PTFE_Tube_4x2:1 — Fluchtend:65, Fluchtend:66
270. 12VDC-1.1875-X-0.375-DELTA-BOX-FAN:1 — Einfügen:196
271. DIN 84 - ersetzt durch DIN EN ISO 1207 M3 x 10:1 — Einfügen:197, Passend:273
272. DIN 84 - ersetzt durch DIN EN ISO 1207 M3 x 10:2 — Einfügen:198, Passend:275
273. DIN 934 - ersetzt durch DIN EN 24032/28673/28674 M3:7 — Passend:273, Passend:274
274. DIN 934 - ersetzt durch DIN EN 24032/28673/28674 M3:8 — Passend:275, Passend:276
275. DIN 84 - ersetzt durch DIN EN ISO 1207 M3 x 22:1 — Einfügen:200, Passend:277
276. DIN 84 - ersetzt durch DIN EN ISO 1207 M3 x 22:2 — Einfügen:199, Passend:279
277. DIN 934 - ersetzt durch DIN EN 24032/28673/28674 M3:9 — Passend:277, Passend:278
278. DIN 934 - ersetzt durch DIN EN 24032/28673/28674 M3:10 — Passend:279, Passend:280
279. DIN 84 - ersetzt durch DIN EN ISO 1207 M3 x 18:1 — Einfügen:202, Passend:283
280. DIN 84 - ersetzt durch DIN EN ISO 1207 M3 x 18:2 — Einfügen:201, Passend:281
281. DIN 934 - ersetzt durch DIN EN 24032/28673/28674 M3:11 — Passend:281, Passend:282
282. DIN 934 - ersetzt durch DIN EN 24032/28673/28674 M3:12 — Passend:283, Passend:284
283. gt2_clip_v2:1 — Passend:285, Fluchtend:67, Fluchtend:68, Passend:286, Passend:295
284. gt2_clip_v2:2 — Passend:289, Fluchtend:73, Fluchtend:74, Passend:291
285. gt2_clip_v2:3 — Passend:288, Fluchtend:71, Fluchtend:72, Passend:297
286. gt2_clip_v2:4 — Passend:287, Fluchtend:69, Fluchtend:70, Passend:293
287. DIN 84 - ersetzt durch DIN EN ISO 1207 M3 x 14:1 — Einfügen:203, Passend:290
288. DIN 84 - ersetzt durch DIN EN ISO 1207 M3 x 14:2 — Einfügen:204, Passend:292
289. DIN 84 - ersetzt durch DIN EN ISO 1207 M3 x 14:3 — Einfügen:205, Passend:294
290. DIN 84 - ersetzt durch DIN EN ISO 1207 M3 x 14:4 — Einfügen:206, Passend:296
291. DIN 934 - ersetzt durch DIN EN 24032/28673/28674 M3:13 — Passend:290, Passend:291
292. DIN 934 - ersetzt durch DIN EN 24032/28673/28674 M3:14 — Passend:292, Passend:293
293. DIN 934 - ersetzt durch DIN EN 24032/28673/28674 M3:15 — Passend:294, Passend:295
294. DIN 934 - ersetzt durch DIN EN 24032/28673/28674 M3:16 — Passend:296, Passend:297
## Relationships (476: Mate 214, Insert 183, Flush 66, Tangent 13)
- Tangential:1: Motedius_20x20_B-Type_Slot-6_500:1 ↔ Motedius_20x20_B-Type_Slot-6_500:2
- Fluchtend:1 [Flush] (20 mm): Motedius_20x20_B-Type_Slot-6_500:1 ↔ Motedius_20x20_B-Type_Slot-6_500:2
- Passend:1 [Mate]: Motedius_20x20_B-Type_Slot-6_500:1 ↔ Motedius_20x20_B-Type_Slot-6_500:2
- Tangential:2: Motedius_20x20_B-Type_Slot-6_500:2 ↔ Motedius_20x20_B-Type_Slot-6_500:3
- Passend:2 [Mate]: Motedius_20x20_B-Type_Slot-6_500:2 ↔ Motedius_20x20_B-Type_Slot-6_500:3
- Fluchtend:2 [Flush] (-20 mm): Motedius_20x20_B-Type_Slot-6_500:2 ↔ Motedius_20x20_B-Type_Slot-6_500:3
- Tangential:3: Motedius_20x20_B-Type_Slot-6_500:1 ↔ Motedius_20x20_B-Type_Slot-6_500:4
- Fluchtend:3 [Flush] (-20 mm): Motedius_20x20_B-Type_Slot-6_500:1 ↔ Motedius_20x20_B-Type_Slot-6_500:4
- Passend:3 [Mate]: Motedius_20x20_B-Type_Slot-6_500:1 ↔ Motedius_20x20_B-Type_Slot-6_500:4
- Passend:4 [Mate] (-250 mm): Motedius_20x20_B-Type_Slot-6_500:4
- Passend:5 [Mate] (-250 mm): Motedius_20x20_B-Type_Slot-6_500:1
- Passend:6 [Mate] (-250 mm): Motedius_20x20_B-Type_Slot-6_500:4
- Passend:7 [Mate]: Motedius_20x20_B-Type_Slot-6_500:1 ↔ Motedius_20x20_B-Type_Slot-6_500:5
- Fluchtend:4 [Flush]: Motedius_20x20_B-Type_Slot-6_500:4 ↔ Motedius_20x20_B-Type_Slot-6_500:5
- Passend:8 [Mate]: Motedius_20x20_B-Type_Slot-6_500:4 ↔ Motedius_20x20_B-Type_Slot-6_500:5
- Passend:9 [Mate]: Motedius_20x20_B-Type_Slot-6_500:1 ↔ Motedius_20x20_B-Type_Slot-6_500:6
- Fluchtend:5 [Flush]: Motedius_20x20_B-Type_Slot-6_500:2 ↔ Motedius_20x20_B-Type_Slot-6_500:6
- Passend:10 [Mate]: Motedius_20x20_B-Type_Slot-6_500:2 ↔ Motedius_20x20_B-Type_Slot-6_500:6
- Passend:11 [Mate]: Motedius_20x20_B-Type_Slot-6_500:3 ↔ Motedius_20x20_B-Type_Slot-6_500:8
- Passend:12 [Mate]: Motedius_20x20_B-Type_Slot-6_500:4 ↔ Motedius_20x20_B-Type_Slot-6_500:8
- Fluchtend:6 [Flush]: Motedius_20x20_B-Type_Slot-6_500:4 ↔ Motedius_20x20_B-Type_Slot-6_500:8
- Passend:13 [Mate]: Motedius_20x20_B-Type_Slot-6_500:2 ↔ Motedius_20x20_B-Type_Slot-6_500:7
- Passend:14 [Mate]: Motedius_20x20_B-Type_Slot-6_500:3 ↔ Motedius_20x20_B-Type_Slot-6_500:7
- Fluchtend:7 [Flush]: Motedius_20x20_B-Type_Slot-6_500:2 ↔ Motedius_20x20_B-Type_Slot-6_500:7
- Passend:15 [Mate] (-250 mm): Motedius_20x20_B-Type_Slot-6_500_MIR:1
- Passend:16 [Mate]: Motedius_20x20_B-Type_Slot-6_500_MIR:1 ↔ Motedius_20x20_B-Type_Slot-6_500_MIR:2
- Fluchtend:8 [Flush] (20 mm): Motedius_20x20_B-Type_Slot-6_500_MIR:1 ↔ Motedius_20x20_B-Type_Slot-6_500_MIR:2
- Tangential:4: Motedius_20x20_B-Type_Slot-6_500_MIR:1 ↔ Motedius_20x20_B-Type_Slot-6_500_MIR:2
- Fluchtend:9 [Flush] (-20 mm): Motedius_20x20_B-Type_Slot-6_500_MIR:2 ↔ Motedius_20x20_B-Type_Slot-6_500_MIR:3
- Passend:17 [Mate]: Motedius_20x20_B-Type_Slot-6_500_MIR:2 ↔ Motedius_20x20_B-Type_Slot-6_500_MIR:3
- Tangential:5: Motedius_20x20_B-Type_Slot-6_500_MIR:2 ↔ Motedius_20x20_B-Type_Slot-6_500_MIR:3
- Passend:18 [Mate] (-250 mm): Motedius_20x20_B-Type_Slot-6_500_MIR:4
- Fluchtend:10 [Flush] (-250 mm): Motedius_20x20_B-Type_Slot-6_500_MIR:4
- Passend:19 [Mate]: Motedius_20x20_B-Type_Slot-6_500_MIR:1 ↔ Motedius_20x20_B-Type_Slot-6_500_MIR:4
- Fluchtend:11 [Flush] (-20 mm): Motedius_20x20_B-Type_Slot-6_500_MIR:1 ↔ Motedius_20x20_B-Type_Slot-6_500_MIR:4
- Tangential:6: Motedius_20x20_B-Type_Slot-6_500_MIR:1 ↔ Motedius_20x20_B-Type_Slot-6_500_MIR:4
- Einfügen:1 [Insert]: Nema17_Schrittmotor:1 ↔ Nema17_Montageplatte:1
- Tangential:7: Nema17_Schrittmotor:1 ↔ Nema17_Montageplatte:1
- Einfügen:2 [Insert] (3 mm): Nema17_Schrittmotor:1 ↔ DIN 84 - ersetzt durch DIN EN ISO 1207 M3 x 6:1
- Einfügen:3 [Insert] (3 mm): Nema17_Schrittmotor:1 ↔ DIN 84 - ersetzt durch DIN EN ISO 1207 M3 x 6:3
- Einfügen:4 [Insert] (3 mm): Nema17_Schrittmotor:1 ↔ DIN 84 - ersetzt durch DIN EN ISO 1207 M3 x 6:4
- Einfügen:5 [Insert] (3 mm): Nema17_Schrittmotor:1 ↔ DIN 84 - ersetzt durch DIN EN ISO 1207 M3 x 6:2
- Passend:20 [Mate]: Motedius_20x20_B-Type_Slot-6_500:5 ↔ Nema17_Montageplatte:1
- Fluchtend:12 [Flush]: Motedius_20x20_B-Type_Slot-6_500:5 ↔ Nema17_Montageplatte:1
- Passend:21 [Mate] (20 mm): Motedius_20x20_B-Type_Slot-6_500_MIR:1 ↔ Nema17_Montageplatte:1
- [Insert]: Nema17_Schrittmotor:2 ↔ Nema17_Montageplatte:2
- [Tangent]: Nema17_Schrittmotor:2 ↔ Nema17_Montageplatte:2
- [Insert] (3 mm): Nema17_Schrittmotor:2 ↔ DIN 84 - ersetzt durch DIN EN ISO 1207 M3 x 6:5
- [Insert] (3 mm): Nema17_Schrittmotor:2 ↔ DIN 84 - ersetzt durch DIN EN ISO 1207 M3 x 6:7
- [Insert] (3 mm): Nema17_Schrittmotor:2 ↔ DIN 84 - ersetzt durch DIN EN ISO 1207 M3 x 6:8
- [Insert] (3 mm): Nema17_Schrittmotor:2 ↔ DIN 84 - ersetzt durch DIN EN ISO 1207 M3 x 6:6
- Passend:22 [Mate] (20 mm): Motedius_20x20_B-Type_Slot-6_500_MIR:1 ↔ Nema17_Montageplatte:2
- Passend:23 [Mate]: Motedius_20x20_B-Type_Slot-6_500:6 ↔ Nema17_Montageplatte:2
- Fluchtend:13 [Flush]: Motedius_20x20_B-Type_Slot-6_500:6 ↔ Nema17_Montageplatte:2
- [Insert]: Nema17_Schrittmotor:3 ↔ Nema17_Montageplatte:3
- [Tangent]: Nema17_Schrittmotor:3 ↔ Nema17_Montageplatte:3
- [Insert] (3 mm): Nema17_Schrittmotor:3 ↔ DIN 84 - ersetzt durch DIN EN ISO 1207 M3 x 6:9
- [Insert] (3 mm): Nema17_Schrittmotor:3 ↔ DIN 84 - ersetzt durch DIN EN ISO 1207 M3 x 6:11
- [Insert] (3 mm): Nema17_Schrittmotor:3 ↔ DIN 84 - ersetzt durch DIN EN ISO 1207 M3 x 6:12
- [Insert] (3 mm): Nema17_Schrittmotor:3 ↔ DIN 84 - ersetzt durch DIN EN ISO 1207 M3 x 6:10
- Passend:24 [Mate] (20 mm): Motedius_20x20_B-Type_Slot-6_500_MIR:3 ↔ Nema17_Montageplatte:3
- Passend:25 [Mate]: Motedius_20x20_B-Type_Slot-6_500:7 ↔ Nema17_Montageplatte:3
- Fluchtend:14 [Flush]: Motedius_20x20_B-Type_Slot-6_500:7 ↔ Nema17_Montageplatte:3
- [Insert]: Nema17_Schrittmotor:4 ↔ Nema17_Montageplatte:4
- [Tangent]: Nema17_Schrittmotor:4 ↔ Nema17_Montageplatte:4
- [Insert] (3 mm): Nema17_Schrittmotor:4 ↔ DIN 84 - ersetzt durch DIN EN ISO 1207 M3 x 6:13
- [Insert] (3 mm): Nema17_Schrittmotor:4 ↔ DIN 84 - ersetzt durch DIN EN ISO 1207 M3 x 6:15
- [Insert] (3 mm): Nema17_Schrittmotor:4 ↔ DIN 84 - ersetzt durch DIN EN ISO 1207 M3 x 6:16
- [Insert] (3 mm): Nema17_Schrittmotor:4 ↔ DIN 84 - ersetzt durch DIN EN ISO 1207 M3 x 6:14
- Passend:26 [Mate] (20 mm): Motedius_20x20_B-Type_Slot-6_500_MIR:3 ↔ Nema17_Montageplatte:4
- Passend:27 [Mate]: Motedius_20x20_B-Type_Slot-6_500:8 ↔ Nema17_Montageplatte:4
- Fluchtend:15 [Flush]: Motedius_20x20_B-Type_Slot-6_500:8 ↔ Nema17_Montageplatte:4
- Passend:52 [Mate]: DIN 84 - ersetzt durch DIN EN ISO 1207 M6 x 50:1 ↔ DIN 125-1 A A 6,4:9
- Passend:53 [Mate]: DIN 84 - ersetzt durch DIN EN ISO 1207 M6 x 50:1 ↔ DIN 125-1 A A 6,4:9
- [Mate]: DIN 84 - M6 x 70:1 ↔ DIN 125-1 A A 6,4:10
- [Mate]: DIN 84 - M6 x 70:1 ↔ DIN 125-1 A A 6,4:10
- [Mate]: DIN 84 - ersetzt durch DIN EN ISO 1207 M6 x 50:3 ↔ DIN 125-1 A A 6,4:11
- [Mate]: DIN 84 - ersetzt durch DIN EN ISO 1207 M6 x 50:3 ↔ DIN 125-1 A A 6,4:11
- [Mate]: DIN 84 - ersetzt durch DIN EN ISO 1207 M6 x 50:4 ↔ DIN 125-1 A A 6,4:12
- [Mate]: DIN 84 - ersetzt durch DIN EN ISO 1207 M6 x 50:4 ↔ DIN 125-1 A A 6,4:12
- Einfügen:25 [Insert] (5.5 mm): Motedius_20x20_B-Type_Slot-6_500_MIR:3 ↔ DIN 125-1 A A 6,4:9
- Einfügen:26 [Insert] (5.5 mm): Motedius_20x20_B-Type_Slot-6_500_MIR:1 ↔ DIN 125-1 A A 6,4:11
- Einfügen:27 [Insert] (5.5 mm): Motedius_20x20_B-Type_Slot-6_500_MIR:1 ↔ DIN 125-1 A A 6,4:12
- Einfügen:28 [Insert] (5.5 mm): Motedius_20x20_B-Type_Slot-6_500_MIR:3 ↔ DIN 125-1 A A 6,4:10
- Passend:62 [Mate]: DIN 84 - ersetzt durch DIN EN ISO 1207 M6 x 50:1 ↔ DIN 125-1 A A 6,4:14
- Passend:63 [Mate]: Motedius_20x20_B-Type_Slot-6_500_MIR:4 ↔ DIN 125-1 A A 6,4:14
- Passend:64 [Mate]: DIN 84 - ersetzt durch DIN EN ISO 1207 M6 x 50:3 ↔ DIN 125-1 A A 6,4:15
- Passend:65 [Mate]: Motedius_20x20_B-Type_Slot-6_500_MIR:4 ↔ DIN 125-1 A A 6,4:15
- Passend:66 [Mate]: DIN 84 - ersetzt durch DIN EN ISO 1207 M6 x 50:4 ↔ DIN 125-1 A A 6,4:16
- Passend:67 [Mate]: Motedius_20x20_B-Type_Slot-6_500_MIR:2 ↔ DIN 125-1 A A 6,4:16
- Passend:70 [Mate]: DIN 84 - ersetzt durch DIN EN ISO 1207 M6 x 50:1 ↔ DIN 934 - ersetzt durch DIN EN 24032/28673/28674 M6:6
- Passend:71 [Mate]: DIN 125-1 A A 6,4:14 ↔ DIN 934 - ersetzt durch DIN EN 24032/28673/28674 M6:6
- Passend:72 [Mate]: DIN 84 - ersetzt durch DIN EN ISO 1207 M6 x 50:3 ↔ DIN 934 - ersetzt durch DIN EN 24032/28673/28674 M6:7
- Passend:73 [Mate]: DIN 125-1 A A 6,4:15 ↔ DIN 934 - ersetzt durch DIN EN 24032/28673/28674 M6:7
- Passend:74 [Mate]: DIN 84 - ersetzt durch DIN EN ISO 1207 M6 x 50:4 ↔ DIN 934 - ersetzt durch DIN EN 24032/28673/28674 M6:8
- Passend:75 [Mate]: DIN 125-1 A A 6,4:16 ↔ DIN 934 - ersetzt durch DIN EN 24032/28673/28674 M6:8
- Passend:76 [Mate]: Motedius_Gelenkfuß_10_PA_M6x60:1 ↔ DIN 125-1 A A 6,4:17
- Passend:77 [Mate]: Motedius_Gelenkfuß_10_PA_M6x60:1 ↔ DIN 125-1 A A 6,4:17
- Einfügen:29 [Insert] (5.5 mm): Motedius_20x20_B-Type_Slot-6_500:4 ↔ DIN 125-1 A A 6,4:17
- Passend:78 [Mate]: Motedius_Gelenkfuß_10_PA_M6x60:1 ↔ DIN 125-1 A A 6,4:18
- Passend:79 [Mate]: Motedius_20x20_B-Type_Slot-6_500:1 ↔ DIN 125-1 A A 6,4:18
- Passend:80 [Mate]: Motedius_Gelenkfuß_10_PA_M6x60:1 ↔ DIN 934 - ersetzt durch DIN EN 24032/28673/28674 M6:9
- Passend:81 [Mate]: DIN 125-1 A A 6,4:18 ↔ DIN 934 - ersetzt durch DIN EN 24032/28673/28674 M6:9